# Autodesk Inventor assembly: Battery_holder
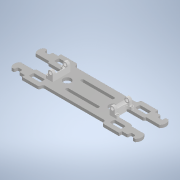
[picture p0: Inventor's stored thumbnail of the model, 180x180]
Saved by Autodesk Inventor 2022 (Build 260153000, 153)
## iProperties
Created: 2023-01-30
Part Number: Battery_holder
Document SubType Name: Assembly
Designer: scott
Author: scott
## Documents named in this file (3)
- C:\Users\scott\OneDrive\Documents\Cat project\Git_repository\Flinders_OpenCat\CAD components\Battery_holder.iam
- C:\Users\scott\OneDrive\Documents\Cat project\Git_repository\Flinders_OpenCat\CAD components\NybbleDIY\Imported Components\BellyPlate\BellyPlate.ipt
- C:\Users\scott\OneDrive\Documents\Cat project\Git_repository\Flinders_OpenCat\CAD components\Imported Components\Battery_holer_lower\Battery_holer_lower.ipt
## Components (3 placed, 2 different names)
1. BellyPlate:1 — Mate:1, Mate:2, Mate:3, Mate:4, Mate:5, Mate:6
2. Battery_holer_lower:1 — Mate:1, Mate:2, Mate:3
3. Battery_holer_lower:2 — Mate:4, Mate:5, Mate:6
## Relationships (6: Mate 6)
- Mate:1: BellyPlate:1 ↔ Battery_holer_lower:1
- Mate:2: BellyPlate:1 ↔ Battery_holer_lower:1
- Mate:3: BellyPlate:1 ↔ Battery_holer_lower:1
- Mate:4: BellyPlate:1 ↔ Battery_holer_lower:2
- Mate:5: BellyPlate:1 ↔ Battery_holer_lower:2
- Mate:6: BellyPlate:1 ↔ Battery_holer_lower:2
